# Autodesk Inventor assembly: Right Side Tower Assembly
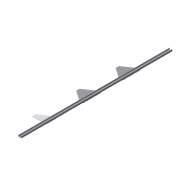
[picture p0: Inventor's stored thumbnail of the model, 180x180]
Saved by Autodesk Inventor 2015 (Build 190159000, 159)
## iProperties
Created: 2015-01-24
Part Number: Right Side Tower Assembly
Document SubType Name: Assembly
Designer: Peter
Author: Peter
## Documents named in this file (4)
- C:\Users\Noah\Desktop\FIRST-Team-1719-CAD-Team\2015 Robot CAD\Lifter Super Structure\Tower\Side-Towers Assemblies\Left Side Tower Assembly.iam
- C:\Users\Noah\Desktop\FIRST-Team-1719-CAD-Team\2015 Robot CAD\Lifter Super Structure\Tower\Side-Towers Assemblies\Vertical-Unistrut-Tower-75.ipt
- C:\Users\Noah\Desktop\FIRST-Team-1719-CAD-Team\2015 Robot CAD\Lifter Super Structure\Tower\Side-Towers Assemblies\Center-Tower-Brace.ipt
- C:\Users\Noah\Desktop\FIRST-Team-1719-CAD-Team\2015 Robot CAD\Lifter Super Structure\Tower\Side-Towers Assemblies\Corner-Tower-Brace.ipt
## Components (4 placed, 3 different names)
1. Vertical-Unistrut-Tower-75:1 — Flush:7, Mate:6, Mate:7, Mate:8, Flush:9, Flush:10, Flush:11, Flush:12
2. Center-Tower-Brace:1 — Mate:8, Flush:9
3. Center-Tower-Brace:2 — Flush:7, Mate:7, Flush:10
4. Corner-Tower-Brace:2 — Mate:6, Flush:11, Flush:12
## Relationships (8: Flush 5, Mate 3)
- Flush:7 (-774.7 mm): Vertical-Unistrut-Tower-75:1 ↔ Center-Tower-Brace:2
- Mate:6: Vertical-Unistrut-Tower-75:1 ↔ Corner-Tower-Brace:2
- Mate:7: Vertical-Unistrut-Tower-75:1 ↔ Center-Tower-Brace:2
- Mate:8: Vertical-Unistrut-Tower-75:1 ↔ Center-Tower-Brace:1
- Flush:9: Vertical-Unistrut-Tower-75:1 ↔ Center-Tower-Brace:1
- Flush:10: Vertical-Unistrut-Tower-75:1 ↔ Center-Tower-Brace:2
- Flush:11: Vertical-Unistrut-Tower-75:1 ↔ Corner-Tower-Brace:2
- Flush:12 (311.15 mm): Vertical-Unistrut-Tower-75:1 ↔ Corner-Tower-Brace:2
## Named parameters: Lower_Center_Tower_Brace_Height = -774.7 mm
